# Autodesk Inventor assembly: axis_7_bottom_frame
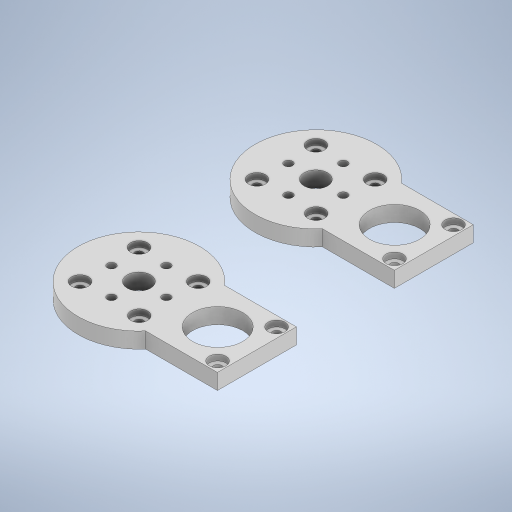
[picture p0: Inventor's stored thumbnail of the model, 512x512]
Saved by Autodesk Inventor 2024.2 (Build 282272000, 272)
## iProperties
Created: 2024-01-07
Part Number: axis_7_bottom_frame
Document SubType Name: Assembly
Designer: chanh
Author: chanh
## Documents named in this file (2)
- C:\Users\chanh\내 드라이브\로봇\Humanoid\Roboin Humanoid Project\Inventor\rh_plus_7_axis_robot_arm_hardware\CAM\4T\axis_7_bottom_frame.iam
- C:\Users\chanh\내 드라이브\로봇\Humanoid\Roboin Humanoid Project\Inventor\rh_plus_7_axis_robot_arm_hardware\CAM\4T\axis_7_bottom_frame.ipt
## Components (2 placed, 1 different names)
1. axis_7_bottom_frame:1 — Mate:1, Flush:1, Flush:2, Mate:3, Flush:3
2. axis_7_bottom_frame:2 — Mate:2, Mate:3, Flush:3
## Relationships (6: Mate 3, Flush 3)
- Mate:1: axis_7_bottom_frame:1
- Flush:1: axis_7_bottom_frame:1
- Flush:2: axis_7_bottom_frame:1
- Mate:2: axis_7_bottom_frame:2
- Mate:3 (25 mm): axis_7_bottom_frame:1 ↔ axis_7_bottom_frame:2
- Flush:3: axis_7_bottom_frame:1 ↔ axis_7_bottom_frame:2
